# Autodesk Inventor assembly: ice-keys-p3
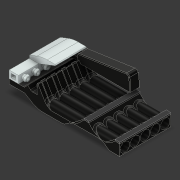
[picture p0: Inventor's stored thumbnail of the model, 180x180]
Saved by Autodesk Inventor 2020.2 (Build 242310000, 310)
## iProperties
Created: 2020-07-06
Part Number: ice-keys-p3
Document SubType Name: Assembly
Designer: isaac
Mass: 15.6119 g
Surface Area: 114.007 cm^2
Volume: 14.7752 cm^3
Density: 1.05662 g/cm^3
Author: isaac
## Documents named in this file (6)
- C:\Users\isaac\Documents\ice-keys\p3\inventor\ice-keys-p3.iam
- C:\Users\isaac\Documents\ice-keys\p3\inventor\postvalve.ipt
- C:\Users\isaac\Documents\ice-keys\p3\inventor\black_key.ipt
- C:\Users\isaac\Documents\ice-keys\p3\inventor\padding_strip.ipt
- C:\Users\isaac\Documents\ice-keys\p3\inventor\manifold_lower.ipt
- C:\Users\isaac\Documents\ice-keys\p3\inventor\manifold_upper.ipt
## Components (6 placed, 4 different names)
1. postvalve:1 — Rigid:1, Rigid:2, Rigid:3, Rotational:1
2. black_key:1 — Rotational:1
3. padding_strip:1 — Rigid:1
4. padding_strip:2 — Rigid:2
5. manifold:1 — Rigid:3, Rigid:4
6. manifold:2 — Rigid:4
## Relationships (5: WeldJoint 4, RevoluteJoint 1)
- Rigid:1 [WeldJoint]: postvalve:1 ↔ padding_strip:1
- Rigid:2 [WeldJoint]: postvalve:1 ↔ padding_strip:2
- Rigid:3 [WeldJoint]: postvalve:1 ↔ manifold:1
- Rigid:4 [WeldJoint]: manifold:1 ↔ manifold:2
- Rotational:1 [RevoluteJoint]: postvalve:1 ↔ black_key:1
